# Autodesk Inventor assembly: TTPS12T5200-A-P5
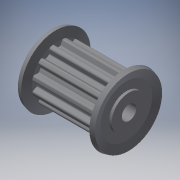
[picture p0: Inventor's stored thumbnail of the model, 180x180]
Saved by Autodesk Inventor 2019 (Build 230136000, 136)
## iProperties
Category: PARTsolutions
Company: MISUMI
Created: 2023-11-09
Part Number: TTPS12T5200-A-P5
Catalog Web Link: www.cadenas.de
Description: TTPA__T5050, TTPA__T5100, TTPA__T5150, TTPA__T5200, TTPA__T5250, TTPB__T5050, TTPB__T5100, TTPB__T5150, TTPB__T5200, TTPB__T5250, TTPK__T5050, TTPK__T5100, TTPK__T5150, TTPK__T5200, TTPK__T5250, TTPN__T5050, TTPN__T5100, TTPN__T5150, TTPN__T5200, TTPN__T5250, TTPT__T5050, TTPT__T5100, TTPT__T5150, TTPT__T5200, TTPT__T5250, TTPM__T5050, TTPM__T5100, TTPM__T5150, TTPM__T5200, TTPM__T5250, TTPP__T5050, TTPP__T5100, TTPP__T5150, TTPP__T5200, TTPP__T5250, TTPS__T5050, TTPS__T5100, TTPS__T5150, TTPS__T5200, TTPS__T5250-Timing Pulleys T5 Type
Vendor: MISUMI
Document SubType Name: Assembly
Designer: psAdmin
Manufacturer: MISUMI
Mass: 5.72212 g
Surface Area: 39.0895 cm^2
Volume: 5.72212 cm^3
Density: 1 g/cm^3
Title: TTPS12T5200-A-P5
Author: Cadenas PARTsolutions
Comments: Timing Pulleys T5 Type
PSOL_IDENT_0: {$CADENAS_DATA/23d-libs/misumi/metric/51_timing_pulleys/ttpt_t5_asmtab.prj},947 {VTYP=3D},{STYP=ASST
PSOL_IDENT_1: AB},{NB=TTPS12T5200-A-P5},{LINA=TTPS12T5200-A-P5},{NN=TTPA__T5050, TTPA__T5100, TTPA__T5150, TTPA__T
PSOL_IDENT_2: 5200, TTPA__T5250, TTPB__T5050, TTPB__T5100, TTPB__T5150, TTPB__T5200, TTPB__T5250, TTPK__T5050, TTP
PSOL_IDENT_3: K__T5100, TTPK__T5150, TTPK__T5200, TTPK__T5250, TTPN__T5050, TTPN__T5100, TTPN__T5150, TTPN__T5200,
PSOL_IDENT_4: TTPN__T5250, TTPT__T5050, TTPT__T5100, TTPT__T5150, TTPT__T5200, TTPT__T5250, TTPM__T5050, TTPM__T5
PSOL_IDENT_5: 100, TTPM__T5150, TTPM__T5200, TTPM__T5250, TTPP__T5050, TTPP__T5100, TTPP__T5150, TTPP__T5200, TTPP
PSOL_IDENT_6: __T5250, TTPS__T5050, TTPS__T5100, TTPS__T5150, TTPS__T5200, TTPS__T5250},{DATE=17.01.2023 09:21:21}
PSOL_IDENT_7: ,{GEOMDATE=17.01.2023 00:45:25},{VERSION=},{LINEID=10},{WBVAR=MATP,ST,TNW,PS,SBS,DD,Z,J,Q,R,S,T,ALT1
PSOL_IDENT_8: ,ALT2,M,QSC,QFC,QTC,ALT3,K,KSC,KFC,KTC,ALT4,ZM,ZSC,ZFC,ZTC,ALT5,ALT6,ALT7,FC,ALT8,SRG,ALT9,BTC,TL,AL
PSOL_IDENT_9: T10,TPC,ALT11,BC,ALT12,SLH,ALT13,BN},{WBNUMERIC=DD,Z,J,Q,R,S,T,QSC,QFC,QTC,K,KSC,KFC,KTC,ZSC,ZFC,ZTC
PSOL_IDENT_10: ,FC,SRG,BTC,TL,BC,SLH,BN}  {NB=TTPS12T5200-A-P5},{LINA=TTPS12T5200-A-P5},{KT=DUMMY},{PN=TTPS12T5200-
PSOL_IDENT_11: A-P5},{TYPE=TTPS},{MATP=SUS304},{MATPALG= 'A2017','Aluminum Alloy 2000 series','S45C','1045 Carbon S
PSOL_IDENT_12: teel Equivalent','SUS304','304 Stainless Steel' },{ST=-},{STALG= '-','-' },{NT=12},{TNW=T5200},{TNWA
PSOL_IDENT_13: LG= 'T5100' , 'T5150' , 'T5200' , 'T5250' },{BW=20},{PS=A},{PSALG= 'A' },{SBS=P},{SBSALG= 'H','Round
PSOL_IDENT_14: Hole','P','Round Hole + Tap','N','New JIS Keywayed Bore + Tap (Standard)','V','Stepped Hole','Y','B
PSOL_IDENT_15: oth Ends Stepped Hole' },{DD=5.00},{DDALG=[5:6/1],6.35,[7:8/1]},{DDHA=[5:6/1],6.35,[7:8/1]},{DDPA=[5
PSOL_IDENT_16: :6/1],6.35,[7:8/1]},{DDNA=[8:8/1]},{DDCA=},{DDVA=[5:6/1]},{DDY=[5:6/1]},{DDWB=},{DDHB=},{DDPB=},{DDN
PSOL_IDENT_17: B=},{DDNK=[10:10/1]},{DDCB=},{DDVFB=},{Z=0},{ZALG=[0]},{ZMIN=7.000},{ZAMAX=8.000},{ZBMAX=0.000},{DDZ=
PSOL_IDENT_18: 5.000},{J=0.0},{JALG=[0]},{JMIN=2.000},{JMAX=25.000},{JPN=},{Q=0},{QALG=[0]},{QRMIN=7.000},{QRMAX=8.
PSOL_IDENT_19: 000},{WBQMIN=9.000},{R=0},{RALG=[0]},{WBRMAX=-2.000},{S=0.0},{SALG=[0]},{SMAX=14.000},{T=0.0},{TALG=
PSOL_IDENT_20: [0]},{TMAX=14.000},{SBSPN=-P5},{A=22},{W=27},{L=0},{PD=19.10},{OD=18.25},{D=0},{DALG=0.000},{DE=12.0
PSOL_IDENT_21: 00},{F=24},{E=12},{TT=1.6},{BBK=0.000},{TTK=0.000},{ALT1=},{ALT1ALG= '','w/o KC90 (Set Screw Angle)'
PSOL_IDENT_22: ,'KC90','with KC90 (Set Screw Angle)' },{ANG=120.000},{ALT1PN=},{ALT2=},{ALT2ALG= '','Not applicable'
PSOL_IDENT_23: },{M=N/A},{MALG= 'N/A' },{MFTALG= 'N/A' },{MSALG= 'N/A' },{M3D=0.000},{KDML=0.000},{ML=0.000},{MUL=
PSOL_IDENT_24: 0.000},{PITCH=0.000},{QSC=0.0},{QSCALG=0},{QFC=0.0},{QFCALG=0},{QTC=0.0},{QTCALG=0},{QPCDMIN=0.000},
PSOL_IDENT_25: {QPCDMINALG=0.000},{QPCDMAX=8.000},{ALT2PN=},{TAP=0.000},{ALT3=},{ALT3ALG= '','Not applicable' },{K=
PSOL_IDENT_26: 0.0},{KALG=0},{KMIN=4.000},{KFTMAX=0.000},{KSMAX=0.000},{KSC=0.0},{KSCALG=0},{KFC=0.0},{KFCALG=0},{K
PSOL_IDENT_27: TC=0.0},{KTCALG=0},{KSCMIN=9.000},{KPCDMIN=9.000},{KPCDMAX=8.000},{ALT3PN=},{ALT4=},{ALT4ALG= '','No
PSOL_IDENT_28: t applicable' },{ALT4MIN=15.500},{ALT4MAX=1.500},{ZM=N/A},{ZMALG= 'N/A' },{ZMFTALG= 'N/A' },{ZMSALG=
PSOL_IDENT_29: 'N/A' },{ZMDD1=0.0},{ZMDD2=0.0},{ZMHH=0.0},{ZSC=0.0},{ZSCALG=[0]},{ZFC=0.0},{ZFCALG=[0]},{ZTC=0.0},
PSOL_IDENT_30: {ZTCALG=[0]},{ZPCDMIN=0.000},{ZPCDMINALG=0.000},{ZPCDMAX=8.000},{ALT4PN=},{ALT5=},{ALT5ALG= '','w/o
PSOL_IDENT_31: Flange not Attached','NFC','with NFC (Flange not Attached)' },{ALT5PN=},{ALT6=},{ALT6ALG= '','w/o Fl
PSOL_IDENT_32: ange Attached on One Side Only','RFC','with RFC (Flange Attached on The Boss Side Only)','LFC','with
PSOL_IDENT_33: LFC (Flange Attached on The Opposite Side Only)' },{ALT6PN=},{ALT7=},{ALT7ALG= '','w/o FC (Flange C
PSOL_IDENT_34: ut)','FC','with FC (Flange Cut)' },{FC=0.0},{FCALG=0},{FCMIN=19.5},{FCMAX=22.0},{ALT7PN=},{ALT8=},{A
PSOL_IDENT_35: LT8ALG= '','Not applicable' },{ALT8ALGALG=8.000},{ALT8DD2=0.000},{ALT8MM=0.000},{ALT8NN=0.000},{QC=0
PSOL_IDENT_36: .000},{KC=0.000},{ZC=0.000},{SRG=0.0},{SRGALG=[0]},{SRGMAX=0.000},{SRGMAX1=0.000},{DD2=0.0},{MM=0.00
PSOL_IDENT_37: },{NN=0.00},{ALT8PN=},{ALT9=},{ALT9ALG= '','Not applicable' },{BTC9=7.000},{TL9=1.000},{BTC=0},{BTCA
PSOL_IDENT_38: LG=[0]},{TL=0.0},{TLALG=0},{TLMIN=1.000},{TLMAX=-27.500},{BTCL=0},{BTCD=0},{ALT9PN=},{WLBCTL=27.000}
PSOL_IDENT_39: ,{ALT10=},{ALT10ALG= '','w/o TPC (Tapped Hole Dimension)','TPC','with TPC (Tapped Hole Dimension)' }
PSOL_IDENT_40: ,{TPC=N/A},{TPCALG= 'N/A' },{TPCM=3.000},{ALT10PN=},{ALT11=},{ALT11ALG= '','Not applicable' },{BC=0.
PSOL_IDENT_41: 0},{BCALG=0},{BCMIN=6.000},{BCMAX=-27.500},{M1WBC=13.500},{ALT11PN=},{KTT=6.625},{ALT12=},{ALT12ALG=
PSOL_IDENT_42: '','w/o SLH (Set Screw Length)','SLH','with SLH (Set Screw Length)' },{SLH=0},{SLHALG=[0]},{ALT12PN=
PSOL_IDENT_43: },{AC=M3x3},{M1=3.000},{M1L=3.000},{ALT13=},{ALT13ALG= '', 'Not applicable' },{BN=0.0},{BNALG=0},{BN
PSOL_IDENT_44: MIN=-26.5},{BNMAX=-17.0},{ALT13PN=},{PPATH=ttpt_t5/ttpa_t5_asmtpl.prj}
NB: TTPS12T5200-A-P5
NN: 0
NT: 12
NBSYN: $PN.
LINA: TTPS12T5200-A-P5
CATALOG: Misumi
PN: TTPS12T5200-A-P5
MATP: 304 Stainless Steel
ST: -
TNW: T5200
BW: 20
PS: A
SBS: Round Hole + Tap
DD: 5
Z: 0
J: 0
Q: 0
R: 0
S: 0
T: 0
A: 22
W: 27
L: 0
PD: 19.1
OD: 18.25
D: 0
F: 24
E: 12
TT: 1.6
ALT1: w/o KC90 (Set Screw Angle)
ALT2: Not applicable
M: N/A
QSC: 0
QFC: 0
QTC: 0
ALT3: Not applicable
K: 0
KSC: 0
KFC: 0
KTC: 0
ALT4: Not applicable
ZM: N/A
ZMDD1: 0
ZMDD2: 0
ZMHH: 0
ZSC: 0
ZFC: 0
ZTC: 0
ALT5: w/o Flange not Attached
ALT6: w/o Flange Attached on One Side Only
ALT7: w/o FC (Flange Cut)
FC: 0
ALT8: Not applicable
SRG: 0
DD2: 0
MM: 0
ALT9: Not applicable
BTC: 0
TL: 0
BTCL: 0
BTCD: 0
ALT10: w/o TPC (Tapped Hole Dimension)
TPC: N/A
ALT11: Not applicable
BC: 0
ALT12: w/o SLH (Set Screw Length)
SLH: 0
AC: M3x3
ALT13: Not applicable
BN: 0
SUPPLIER: MISUMI
ARTICLENO: TTPS12T5200-A-P5
BOMINFO: TTPS12T5200-A-P5
CREATOR: CADENAS GmbH
## Documents named in this file (3)
- e:\temp\worker_COMMON_2\temp\tmp_4572_110_iw01p\format_0\TTPS12T5200-A-P5.iam
- e:\temp\worker_COMMON_2\temp\tmp_4572_110_iw01p\format_0\TTPS12T5200-A-P5_b.ipt
- e:\temp\worker_COMMON_2\temp\tmp_4572_110_iw01p\format_0\SET-SCREW3-3.ipt
## Components (3 placed, 2 different names)
1. TTPS12T5200-A-P5_b:1 — to_screw1_Z@1 <-> CP_Z@2, to_screw2_Z@1 <-> CP_Z@3
2. SET-SCREW3-3:1 — to_screw1_Z@1 <-> CP_Z@2
3. SET-SCREW3-3:2 — to_screw2_Z@1 <-> CP_Z@3
## Relationships (2: Mate 2)
- to_screw1_Z@1 <-> CP_Z@2 [Mate]: TTPS12T5200-A-P5_b:1 ↔ SET-SCREW3-3:1
- to_screw2_Z@1 <-> CP_Z@3 [Mate]: TTPS12T5200-A-P5_b:1 ↔ SET-SCREW3-3:2
